# Autodesk Inventor assembly: High Strength Chain Generator
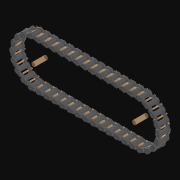
[picture p0: Inventor's stored thumbnail of the model, 180x180]
Saved by Autodesk Inventor 2021 (Build 250183000, 183)
## iProperties
RuleStatus: InUse
Created: 2020-07-07
Part Number: High Strength Chain Generator
Document SubType Name: Assembly
Designer: yuany
AfterDocOpen0: Open Form
Author: yuany
## Documents named in this file (10)
- E:\VEX Cad\Library 1.2\Motion\Chain + Tank Tread\Parametric\High Strength Chain Generator.iam
- E:\VEX Cad\Library 1.1\Motion\Chain + Tank Tread\Parametric\Workpoint Pattern.ipt
- E:\VEX Cad\Library 1.1\Motion\Chain + Tank Tread\High Strength Chain Link.ipt
- E:\VEX Cad\Library 1.1\Motion\Chain + Tank Tread\Tank Tread Traction Link.ipt
- E:\VEX Cad\Library 1.1\Motion\Chain + Tank Tread\Tread Link.ipt
- E:\VEX Cad\Library 1.1\Motion\Chain + Tank Tread\Chain Attachment Link.ipt
- E:\VEX Cad\Library 1.1\Motion\Chain + Tank Tread\Short Flap.ipt
- E:\VEX Cad\Library 1.1\Motion\Chain + Tank Tread\Medium Flap.ipt
- E:\VEX Cad\Library 1.1\Motion\Chain + Tank Tread\Tall Flap.ipt
- E:\VEX Cad\Library 1.1\Motion\Chain + Tank Tread\Parametric\Workpoint Pattern with Slack.ipt
## Components (309 placed, 8 different names)
1. Workpoint Pattern:3 — Mate:1, Mate:2, Mate:3
2. High Strength Chain Link:1 — Mate:1, Mate:2, Mate:3, Flush:1, Mate:4, Angle:1
3. High Strength Chain Link:2
4. High Strength Chain Link:3
5. High Strength Chain Link:4
6. High Strength Chain Link:5
7. High Strength Chain Link:6
8. High Strength Chain Link:7
9. High Strength Chain Link:8
10. High Strength Chain Link:9
11. High Strength Chain Link:10
12. High Strength Chain Link:11
13. High Strength Chain Link:12
14. High Strength Chain Link:13
15. High Strength Chain Link:14
16. High Strength Chain Link:15
17. High Strength Chain Link:16
18. High Strength Chain Link:17
19. High Strength Chain Link:18
20. High Strength Chain Link:19
21. High Strength Chain Link:20
22. High Strength Chain Link:21
23. High Strength Chain Link:22
24. High Strength Chain Link:23
25. High Strength Chain Link:24
26. High Strength Chain Link:25
27. High Strength Chain Link:26
28. High Strength Chain Link:27
29. High Strength Chain Link:28
30. High Strength Chain Link:29
31. High Strength Chain Link:30
32. High Strength Chain Link:31
33. High Strength Chain Link:32
34. High Strength Chain Link:33
35. High Strength Chain Link:34
36. High Strength Chain Link:35
37. High Strength Chain Link:36
38. High Strength Chain Link:37
39. High Strength Chain Link:38
40. High Strength Chain Link:39
41. High Strength Chain Link:40
42. High Strength Chain Link:41
43. High Strength Chain Link:42
44. High Strength Chain Link:43
45. High Strength Chain Link:44
46. Tank Tread Traction Link:1 — Flush:1, Mate:4, Angle:1, Flush:2, Mate:5, Angle:2
47. Tank Tread Traction Link:2
48. Tank Tread Traction Link:3
49. Tank Tread Traction Link:4
50. Tank Tread Traction Link:5
51. Tank Tread Traction Link:6
52. Tank Tread Traction Link:7
53. Tank Tread Traction Link:8
54. Tank Tread Traction Link:9
55. Tank Tread Traction Link:10
56. Tank Tread Traction Link:11
57. Tank Tread Traction Link:12
58. Tank Tread Traction Link:13
59. Tank Tread Traction Link:14
60. Tank Tread Traction Link:15
61. Tank Tread Traction Link:16
62. Tank Tread Traction Link:17
63. Tank Tread Traction Link:18
64. Tank Tread Traction Link:19
65. Tank Tread Traction Link:20
66. Tank Tread Traction Link:21
67. Tank Tread Traction Link:22
68. Tank Tread Traction Link:23
69. Tank Tread Traction Link:24
70. Tank Tread Traction Link:25
71. Tank Tread Traction Link:26
72. Tank Tread Traction Link:27
73. Tank Tread Traction Link:28
74. Tank Tread Traction Link:29
75. Tank Tread Traction Link:30
76. Tank Tread Traction Link:31
77. Tank Tread Traction Link:32
78. Tank Tread Traction Link:33
79. Tank Tread Traction Link:34
80. Tank Tread Traction Link:35
81. Tank Tread Traction Link:36
82. Tank Tread Traction Link:37
83. Tank Tread Traction Link:38
84. Tank Tread Traction Link:39
85. Tank Tread Traction Link:40
86. Tank Tread Traction Link:41
87. Tank Tread Traction Link:42
88. Tank Tread Traction Link:43
89. Tank Tread Traction Link:44
90. Tread Link:1 — Flush:2, Mate:5, Angle:2, Flush:3, Mate:6, Angle:3
91. Tread Link:2
92. Tread Link:3
93. Tread Link:4
94. Tread Link:5
95. Tread Link:6
96. Tread Link:7
97. Tread Link:8
98. Tread Link:9
99. Tread Link:10
100. Tread Link:11
101. Tread Link:12
102. Tread Link:13
103. Tread Link:14
104. Tread Link:15
105. Tread Link:16
106. Tread Link:17
107. Tread Link:18
108. Tread Link:19
109. Tread Link:20
110. Tread Link:21
111. Tread Link:22
112. Tread Link:23
113. Tread Link:24
114. Tread Link:25
115. Tread Link:26
116. Tread Link:27
117. Tread Link:28
118. Tread Link:29
119. Tread Link:30
120. Tread Link:31
121. Tread Link:32
122. Tread Link:33
123. Tread Link:34
124. Tread Link:35
125. Tread Link:36
126. Tread Link:37
127. Tread Link:38
128. Tread Link:39
129. Tread Link:40
130. Tread Link:41
131. Tread Link:42
132. Tread Link:43
133. Tread Link:44
134. Chain Attachment Link:1 — Flush:3, Mate:6, Angle:3
135. Chain Attachment Link:2
136. Chain Attachment Link:3
137. Chain Attachment Link:4
138. Chain Attachment Link:5
139. Chain Attachment Link:6
140. Chain Attachment Link:7
141. Chain Attachment Link:8
142. Chain Attachment Link:9
143. Chain Attachment Link:10
144. Chain Attachment Link:11
145. Chain Attachment Link:12
146. Chain Attachment Link:13
147. Chain Attachment Link:14
148. Chain Attachment Link:15
149. Chain Attachment Link:16
150. Chain Attachment Link:17
151. Chain Attachment Link:18
152. Chain Attachment Link:19
153. Chain Attachment Link:20
154. Chain Attachment Link:21
155. Chain Attachment Link:22
156. Chain Attachment Link:23
157. Chain Attachment Link:24
158. Chain Attachment Link:25
159. Chain Attachment Link:26
160. Chain Attachment Link:27
161. Chain Attachment Link:28
162. Chain Attachment Link:29
163. Chain Attachment Link:30
164. Chain Attachment Link:31
165. Chain Attachment Link:32
166. Chain Attachment Link:33
167. Chain Attachment Link:34
168. Chain Attachment Link:35
169. Chain Attachment Link:36
170. Chain Attachment Link:37
171. Chain Attachment Link:38
172. Chain Attachment Link:39
173. Chain Attachment Link:40
174. Chain Attachment Link:41
175. Chain Attachment Link:42
176. Chain Attachment Link:43
177. Chain Attachment Link:44
178. Short Flap:1 [sub-assembly]
179. Short Flap:2 [sub-assembly]
180. Short Flap:3 [sub-assembly]
181. Short Flap:4 [sub-assembly]
182. Short Flap:5 [sub-assembly]
183. Short Flap:6 [sub-assembly]
184. Short Flap:7 [sub-assembly]
185. Short Flap:8 [sub-assembly]
186. Short Flap:9 [sub-assembly]
187. Short Flap:10 [sub-assembly]
188. Short Flap:11 [sub-assembly]
189. Short Flap:12 [sub-assembly]
190. Short Flap:13 [sub-assembly]
191. Short Flap:14 [sub-assembly]
192. Short Flap:15 [sub-assembly]
193. Short Flap:16 [sub-assembly]
194. Short Flap:17 [sub-assembly]
195. Short Flap:18 [sub-assembly]
196. Short Flap:19 [sub-assembly]
197. Short Flap:20 [sub-assembly]
198. Short Flap:21 [sub-assembly]
199. Short Flap:22 [sub-assembly]
200. Short Flap:23 [sub-assembly]
201. Short Flap:24 [sub-assembly]
202. Short Flap:25 [sub-assembly]
203. Short Flap:26 [sub-assembly]
204. Short Flap:27 [sub-assembly]
205. Short Flap:28 [sub-assembly]
206. Short Flap:29 [sub-assembly]
207. Short Flap:30 [sub-assembly]
208. Short Flap:31 [sub-assembly]
209. Short Flap:32 [sub-assembly]
210. Short Flap:33 [sub-assembly]
211. Short Flap:34 [sub-assembly]
212. Short Flap:35 [sub-assembly]
213. Short Flap:36 [sub-assembly]
214. Short Flap:37 [sub-assembly]
215. Short Flap:38 [sub-assembly]
216. Short Flap:39 [sub-assembly]
217. Short Flap:40 [sub-assembly]
218. Short Flap:41 [sub-assembly]
219. Short Flap:42 [sub-assembly]
220. Short Flap:43 [sub-assembly]
221. Short Flap:44 [sub-assembly]
222. Medium Flap:1 [sub-assembly]
223. Medium Flap:2 [sub-assembly]
224. Medium Flap:3 [sub-assembly]
225. Medium Flap:4 [sub-assembly]
226. Medium Flap:5 [sub-assembly]
227. Medium Flap:6 [sub-assembly]
228. Medium Flap:7 [sub-assembly]
229. Medium Flap:8 [sub-assembly]
230. Medium Flap:9 [sub-assembly]
231. Medium Flap:10 [sub-assembly]
232. Medium Flap:11 [sub-assembly]
233. Medium Flap:12 [sub-assembly]
234. Medium Flap:13 [sub-assembly]
235. Medium Flap:14 [sub-assembly]
236. Medium Flap:15 [sub-assembly]
237. Medium Flap:16 [sub-assembly]
238. Medium Flap:17 [sub-assembly]
239. Medium Flap:18 [sub-assembly]
240. Medium Flap:19 [sub-assembly]
241. Medium Flap:20 [sub-assembly]
242. Medium Flap:21 [sub-assembly]
243. Medium Flap:22 [sub-assembly]
244. Medium Flap:23 [sub-assembly]
245. Medium Flap:24 [sub-assembly]
246. Medium Flap:25 [sub-assembly]
247. Medium Flap:26 [sub-assembly]
248. Medium Flap:27 [sub-assembly]
249. Medium Flap:28 [sub-assembly]
250. Medium Flap:29 [sub-assembly]
251. Medium Flap:30 [sub-assembly]
252. Medium Flap:31 [sub-assembly]
253. Medium Flap:32 [sub-assembly]
254. Medium Flap:33 [sub-assembly]
255. Medium Flap:34 [sub-assembly]
256. Medium Flap:35 [sub-assembly]
257. Medium Flap:36 [sub-assembly]
258. Medium Flap:37 [sub-assembly]
259. Medium Flap:38 [sub-assembly]
260. Medium Flap:39 [sub-assembly]
261. Medium Flap:40 [sub-assembly]
262. Medium Flap:41 [sub-assembly]
263. Medium Flap:42 [sub-assembly]
264. Medium Flap:43 [sub-assembly]
265. Medium Flap:44 [sub-assembly]
266. Tall Flap:1 [sub-assembly]
267. Tall Flap:2 [sub-assembly]
268. Tall Flap:3 [sub-assembly]
269. Tall Flap:4 [sub-assembly]
270. Tall Flap:5 [sub-assembly]
271. Tall Flap:6 [sub-assembly]
272. Tall Flap:7 [sub-assembly]
273. Tall Flap:8 [sub-assembly]
274. Tall Flap:9 [sub-assembly]
275. Tall Flap:10 [sub-assembly]
276. Tall Flap:11 [sub-assembly]
277. Tall Flap:12 [sub-assembly]
278. Tall Flap:13 [sub-assembly]
279. Tall Flap:14 [sub-assembly]
280. Tall Flap:15 [sub-assembly]
281. Tall Flap:16 [sub-assembly]
282. Tall Flap:17 [sub-assembly]
283. Tall Flap:18 [sub-assembly]
284. Tall Flap:19 [sub-assembly]
285. Tall Flap:20 [sub-assembly]
286. Tall Flap:21 [sub-assembly]
287. Tall Flap:22 [sub-assembly]
288. Tall Flap:23 [sub-assembly]
289. Tall Flap:24 [sub-assembly]
290. Tall Flap:25 [sub-assembly]
291. Tall Flap:26 [sub-assembly]
292. Tall Flap:27 [sub-assembly]
293. Tall Flap:28 [sub-assembly]
294. Tall Flap:29 [sub-assembly]
295. Tall Flap:30 [sub-assembly]
296. Tall Flap:31 [sub-assembly]
297. Tall Flap:32 [sub-assembly]
298. Tall Flap:33 [sub-assembly]
299. Tall Flap:34 [sub-assembly]
300. Tall Flap:35 [sub-assembly]
301. Tall Flap:36 [sub-assembly]
302. Tall Flap:37 [sub-assembly]
303. Tall Flap:38 [sub-assembly]
304. Tall Flap:39 [sub-assembly]
305. Tall Flap:40 [sub-assembly]
306. Tall Flap:41 [sub-assembly]
307. Tall Flap:42 [sub-assembly]
308. Tall Flap:43 [sub-assembly]
309. Tall Flap:44 [sub-assembly]
## Component patterns: Chain (44 elements), Traction (44 elements), Tread (44 elements), Chain Attachment (44 elements), Short Flaps (44 elements), Medium Flaps (44 elements), Tall Flaps (44 elements)
## Relationships (12: Mate 6, Flush 3, Angle 3)
- Mate:1: Workpoint Pattern:3 ↔ High Strength Chain Link:1
- Mate:2 (11.938 mm): Workpoint Pattern:3 ↔ High Strength Chain Link:1
- Mate:3: Workpoint Pattern:3 ↔ High Strength Chain Link:1
- Flush:1: High Strength Chain Link:1 ↔ Tank Tread Traction Link:1
- Mate:4: High Strength Chain Link:1 ↔ Tank Tread Traction Link:1
- Angle:1 (180 deg): High Strength Chain Link:1 ↔ Tank Tread Traction Link:1
- Flush:2: Tank Tread Traction Link:1 ↔ Tread Link:1
- Mate:5: Tank Tread Traction Link:1 ↔ Tread Link:1
- Angle:2 (0 deg): Tank Tread Traction Link:1 ↔ Tread Link:1
- Flush:3: Tread Link:1 ↔ Chain Attachment Link:1
- Mate:6: Tread Link:1 ↔ Chain Attachment Link:1
- Angle:3 (0 deg): Tread Link:1 ↔ Chain Attachment Link:1
## Named parameters: Center_Distance = 127 mm, Sprocket1 = 56.388 mm, Sprocket2 = 56.388 mm, CenterDistance = 127 mm, d5_1 = 126.66116 mm, d6_1 = 126.66116 mm, d7_1 = 84.45407 mm, d8_1 = 123.17453 mm
